# Autodesk Inventor assembly: mg996r 3mm leg
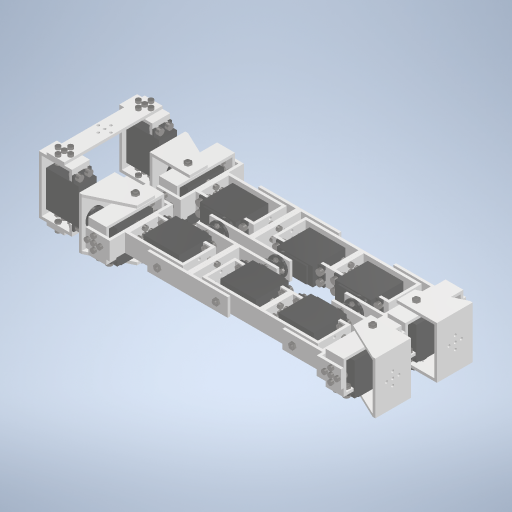
[picture p0: Inventor's stored thumbnail of the model, 512x512]
Saved by Autodesk Inventor 2023 (Build 270158000, 158)
## iProperties
Created: 2022-06-29
Part Number: mg996r 3mm leg
Document SubType Name: Assembly
Designer: isamu
Author: isamu
## Documents named in this file (6)
- D:\personal_projects\robot\inventor\mg996r 3mm leg.iam
- D:\personal_projects\robot\inventor\mg996r left leg bottom middle.iam
- D:\personal_projects\robot\inventor\mg996r leg top.iam
- D:\personal_projects\robot\exports\frames\m2x8.ipt
- D:\personal_projects\robot\exports\frames\m2 nuts.ipt
- D:\personal_projects\robot\inventor\mg996r left leg bottom middle_MIR.iam
## Components (11 placed, 5 different names)
1. mg996r left leg bottom middle:1 [sub-assembly] — Insert:1, Insert:2, Insert:3, Insert:4, Mate:1
2. mg996r leg top:1 [sub-assembly] — Mate:1, Mate:2, Mate:3, Insert:5, Insert:6, Insert:7, Insert:8, Mate:4, Mate:5, Mate:6
3. m2x8:1 — Insert:1, Mate:2
4. m2x8:2 — Insert:4
5. m2x8:3 — Insert:3
6. m2x8:4 — Insert:2, Mate:3
7. m2 nuts:1 — Insert:6
8. m2 nuts:2 — Insert:5
9. m2 nuts:3 — Insert:8
10. m2 nuts:4 — Insert:7
11. mg996r left leg bottom middle_MIR:1 [sub-assembly] — Mate:4, Mate:5, Mate:6
## Relationships (14: Insert 8, Mate 6)
- Insert:1: mg996r left leg bottom middle:1 ↔ m2x8:1
- Insert:2: mg996r left leg bottom middle:1 ↔ m2x8:4
- Insert:3: mg996r left leg bottom middle:1 ↔ m2x8:3
- Insert:4: mg996r left leg bottom middle:1 ↔ m2x8:2
- Mate:1: mg996r left leg bottom middle:1 ↔ mg996r leg top:1
- Mate:2: mg996r leg top:1 ↔ m2x8:1
- Mate:3: mg996r leg top:1 ↔ m2x8:4
- Insert:5: mg996r leg top:1 ↔ m2 nuts:2
- Insert:6: mg996r leg top:1 ↔ m2 nuts:1
- Insert:7: mg996r leg top:1 ↔ m2 nuts:4
- Insert:8: mg996r leg top:1 ↔ m2 nuts:3
- Mate:4: mg996r leg top:1 ↔ mg996r left leg bottom middle_MIR:1
- Mate:5: mg996r leg top:1 ↔ mg996r left leg bottom middle_MIR:1
- Mate:6: mg996r leg top:1 ↔ mg996r left leg bottom middle_MIR:1
